# Autodesk Inventor assembly: platform_0606_fig2_ratio10
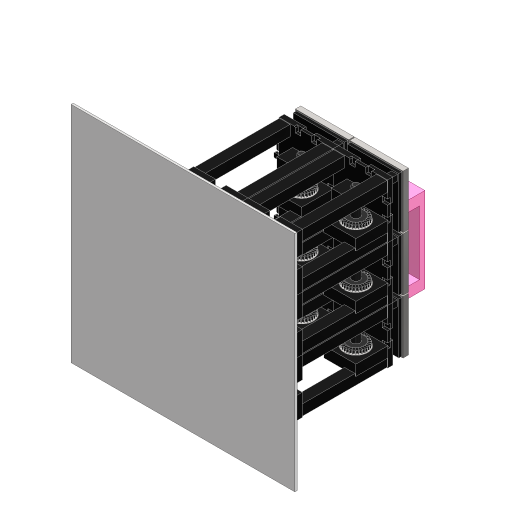
[picture p0: Inventor's stored thumbnail of the model, 512x512]
Saved by Autodesk Inventor 2024 (Build 280153000, 153)
## iProperties
Created: 2024-06-06
Part Number: platform_0606_fig2_ratio10
Document SubType Name: Assembly
Designer: admin
Author: admin
## Documents named in this file (8)
- C:\Users\admin\OneDrive\文件\碩士研究\prototype\plane_unit_0606\platform_0606_fig2_ratio10.iam
- C:\Users\admin\OneDrive\文件\碩士研究\prototype\plane_unit_0606\one_way_bearing.ipt
- C:\Users\admin\OneDrive\文件\碩士研究\prototype\plane_unit_0606\printer_base_plane.ipt
- C:\Users\admin\OneDrive\文件\碩士研究\prototype\plane_unit_0606\rod_1221.ipt
- C:\Users\admin\OneDrive\文件\碩士研究\prototype\plane_unit_0606\iron_plate.ipt
- C:\Users\admin\OneDrive\文件\碩士研究\prototype\plane_unit_0606\plane_unit_1121.ipt
- C:\Users\admin\OneDrive\文件\碩士研究\prototype\plane_unit_0606\gear_pin_1222_.ipt
- C:\Users\admin\OneDrive\文件\碩士研究\prototype\plane_unit_0606\bridge_rect_final_10.ipt
## Components (82 placed, 7 different names)
1. printer_base_plane:1 — 貼合:1, 齊平:1, 齊平:2, 齊平:4, 齊平:5, 齊平:6, 貼合:12
2. bridge_rect_final_10:1 — 齊平:5, 齊平:6, 貼合:12
3. iron_plate:1 — 貼合:9, 貼合:10, 貼合:11, 齊平:4
4. rod_1221:1 — 貼合:7, 貼合:8, 貼合:9, 貼合:10, 貼合:11
5. gear_pin_1222_:1 — 貼合:3, 貼合:4
6. plane_unit_1121:1 — 貼合:1, 齊平:1, 齊平:2, 貼合:2, 齊平:3, 貼合:7, 貼合:8
7. one_way_bearing:1 — 貼合:2, 齊平:3, 貼合:3, 貼合:4
8. iron_plate:2
9. rod_1221:2
10. gear_pin_1222_:2
11. plane_unit_1121:2
12. one_way_bearing:2
13. iron_plate:3
14. rod_1221:3
15. gear_pin_1222_:3
16. plane_unit_1121:3
17. one_way_bearing:3
18. iron_plate:4
19. rod_1221:4
20. gear_pin_1222_:4
21. plane_unit_1121:4
22. one_way_bearing:4
23. iron_plate:5
24. rod_1221:5
25. gear_pin_1222_:5
26. plane_unit_1121:5
27. one_way_bearing:5
28. iron_plate:6
29. rod_1221:6
30. gear_pin_1222_:6
31. plane_unit_1121:6
32. one_way_bearing:6
33. iron_plate:7
34. rod_1221:7
35. gear_pin_1222_:7
36. plane_unit_1121:7
37. one_way_bearing:7
38. iron_plate:8
39. rod_1221:8
40. gear_pin_1222_:8
41. plane_unit_1121:8
42. one_way_bearing:8
43. iron_plate:9
44. rod_1221:9
45. gear_pin_1222_:9
46. plane_unit_1121:9
47. one_way_bearing:9
48. iron_plate:10
49. rod_1221:10
50. gear_pin_1222_:10
51. plane_unit_1121:10
52. one_way_bearing:10
53. iron_plate:11
54. rod_1221:11
55. gear_pin_1222_:11
56. plane_unit_1121:11
57. one_way_bearing:11
58. iron_plate:12
59. rod_1221:12
60. gear_pin_1222_:12
61. plane_unit_1121:12
62. one_way_bearing:12
63. iron_plate:13
64. rod_1221:13
65. gear_pin_1222_:13
66. plane_unit_1121:13
67. one_way_bearing:13
68. iron_plate:14
69. rod_1221:14
70. gear_pin_1222_:14
71. plane_unit_1121:14
72. one_way_bearing:14
73. iron_plate:15
74. rod_1221:15
75. gear_pin_1222_:15
76. plane_unit_1121:15
77. one_way_bearing:15
78. iron_plate:16
79. rod_1221:16
80. gear_pin_1222_:16
81. plane_unit_1121:16
82. one_way_bearing:16
## Component patterns: (16 elements, first: iron_plate:1 + rod_1221:1 + gear_pin_1222_:1 + plane_unit_1121:1 + one_way_bearing:1)
## Relationships (16: Mate 10, Flush 6)
- 貼合:1 [Mate]: printer_base_plane:1 ↔ plane_unit_1121:1
- 齊平:1 [Flush] (5 mm): printer_base_plane:1 ↔ plane_unit_1121:1
- 齊平:2 [Flush] (5 mm): printer_base_plane:1 ↔ plane_unit_1121:1
- 貼合:2 [Mate]: plane_unit_1121:1 ↔ one_way_bearing:1
- 齊平:3 [Flush]: plane_unit_1121:1 ↔ one_way_bearing:1
- 貼合:3 [Mate]: gear_pin_1222_:1 ↔ one_way_bearing:1
- 貼合:4 [Mate]: gear_pin_1222_:1 ↔ one_way_bearing:1
- 貼合:7 [Mate] (0.2 mm): rod_1221:1 ↔ plane_unit_1121:1
- 貼合:8 [Mate] (0.2 mm): rod_1221:1 ↔ plane_unit_1121:1
- 貼合:9 [Mate]: iron_plate:1 ↔ rod_1221:1
- 貼合:10 [Mate]: iron_plate:1 ↔ rod_1221:1
- 貼合:11 [Mate]: iron_plate:1 ↔ rod_1221:1
- 齊平:4 [Flush] (-110 mm): printer_base_plane:1 ↔ iron_plate:1
- 齊平:5 [Flush] (15 mm): printer_base_plane:1 ↔ bridge_rect_final_10:1
- 齊平:6 [Flush] (41 mm): printer_base_plane:1 ↔ bridge_rect_final_10:1
- 貼合:12 [Mate] (110 mm): printer_base_plane:1 ↔ bridge_rect_final_10:1
